# Autodesk Inventor assembly: 4in omni connected to gear
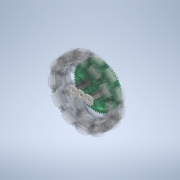
[picture p0: Inventor's stored thumbnail of the model, 180x180]
Saved by Autodesk Inventor 2022.2 (Build 262287010, 287A)
## iProperties
Created: 2022-05-25
Part Number: 4in omni connected to gear
Document SubType Name: Assembly
Designer: Main Account
Author: Main Account
## Documents named in this file (8)
- D:\Documents\Inventor\VEX\Projects\SpinUpPrototypes\4in omni connected to gear.iam
- D:\Documents\Inventor\VEX\Library Backup\Library 1.3\Motion\Gears\HS 60T Gear, Circle.ipt
- D:\Documents\Inventor\VEX\Library Backup\Library 1.3\Motion\Wheels\Omnis\4 Omni, Circle.ipt
- D:\Documents\Inventor\VEX\Library Backup\Library 1.3\Structure\Standoff\Standoff 1.00.ipt
- D:\Documents\Inventor\VEX\Library Backup\Library 1.3\Structure\Standoff.ipt
- D:\Documents\Inventor\VEX\Library Backup\Library 1.3\Structure\Plates\Aluminum\VEX Plates\Alu Plate VEX 1x3.ipt
- D:\Documents\Inventor\VEX\Library Backup\Library 1.3\Motion\Spacers\Washer Steel\SWasher .375 OD x .031250.ipt
- D:\Documents\Inventor\VEX\Library Backup\Library 1.3\Motion\Spacers\Washer Steel.ipt
## Components (6 placed, 5 different names)
1. HS 60T Gear, Circle:1 — Mate:1, Insert:1, Insert:2, Rotation:1
2. 4 Omni, Circle:1 — Mate:1, Rotation:1, Insert:5
3. Standoff 1.00:1 — Insert:1, Insert:4
4. Standoff 1.00:2 — Insert:2, Insert:3
5. Alu Plate VEX 1x3:1 — Insert:3, Insert:4, Mate:2
6. SWasher .375 OD x .031250:1 — Insert:5, Mate:2
## Relationships (8: Insert 5, Mate 2, RelateRotation 1)
- Mate:1: HS 60T Gear, Circle:1 ↔ 4 Omni, Circle:1
- Insert:1: HS 60T Gear, Circle:1 ↔ Standoff 1.00:1
- Insert:2: HS 60T Gear, Circle:1 ↔ Standoff 1.00:2
- Rotation:1 [RelateRotation] (1 ul): HS 60T Gear, Circle:1 ↔ 4 Omni, Circle:1
- Insert:3: Standoff 1.00:2 ↔ Alu Plate VEX 1x3:1
- Insert:4: Standoff 1.00:1 ↔ Alu Plate VEX 1x3:1
- Insert:5: 4 Omni, Circle:1 ↔ SWasher .375 OD x .031250:1
- Mate:2: Alu Plate VEX 1x3:1 ↔ SWasher .375 OD x .031250:1
